# Autodesk Inventor assembly: oar_buttons
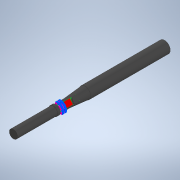
[picture p0: Inventor's stored thumbnail of the model, 180x180]
Saved by Autodesk Inventor 2020 (Build 240168000, 168)
## iProperties
Created: 2019-11-15
Part Number: oar_buttons
Document SubType Name: Assembly
Designer: suchanek
Author: suchanek
## Documents named in this file (3)
- D:\suchanek\programming\rowing_steering\model_final\oar_buttons1.iam
- D:\suchanek\programming\rowing_steering\model_final\oar.ipt
- D:\suchanek\programming\rowing_steering\model_final\buttons1.iam
## Components (2 placed, 2 different names)
1. oar:1 — Rotational:1
2. buttons1:1 [sub-assembly] — Rotational:1
## Relationships (1: RevoluteJoint 1)
- Rotational:1 [RevoluteJoint]: oar:1 ↔ buttons1:1
